# Autodesk Inventor assembly: ASY TKS 3510 Central collector
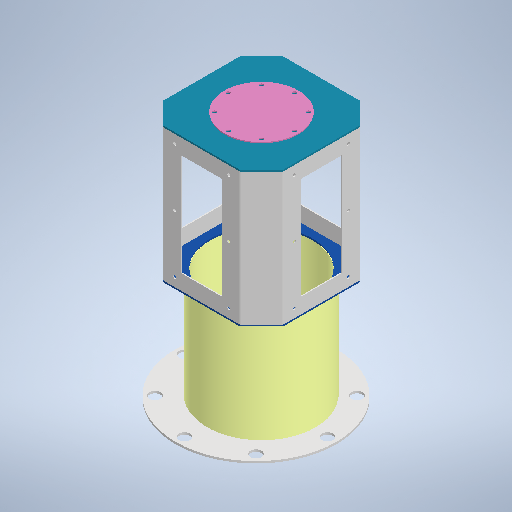
[picture p0: Inventor's stored thumbnail of the model, 512x512]
Saved by Autodesk Inventor 2025 (Build 290162010, 162A)
## iProperties
Created: 2025-07-21
Part Number: ASY TKS 3510 Central collector
Document SubType Name: Assembly
Designer: admin
Author: admin
## Documents named in this file (7)
- C:\Users\pokla\Documents\Inventor\ANP--Antipayuta\FDS 1400\ASY TKS 3510 Central collector.iam
- C:\Users\pokla\Documents\Inventor\ANP--Antipayuta\FDS 1400\ANP 1411 BOTTOM DS main flange.ipt
- C:\Users\pokla\Documents\Inventor\ANP--Antipayuta\FDS 1400\ANP 1452 BOTTOM DS main tube.ipt
- C:\Users\pokla\Documents\Inventor\ANP--Antipayuta\FDS 1400\ANP 1453 BOTTOM DS reduce flange.ipt
- C:\Users\pokla\Documents\Inventor\ANP--Antipayuta\FDS 1400\ANP 1454 BOTTOM DS box wall 1.ipt
- C:\Users\pokla\Documents\Inventor\ANP--Antipayuta\FDS 1400\ANP 1455 BOTTOM DS cup.ipt
- C:\Users\pokla\Documents\Inventor\ANP--Antipayuta\FDS 1400\ANP 1456 BOTTOM DS cup plug.ipt
## Components (7 placed, 6 different names)
1. ANP 1411 BOTTOM DS main flange.ipt:1
2. ANP 1452 BOTTOM DS main tube.ipt:1 — Rigid:6
3. ANP 1453 BOTTOM DS reduce flange.ipt:1 — Rigid:2, Rigid:3, Rigid:6
4. ANP 1454 BOTTOM DS box wall 1.ipt:1 — Rigid:3
5. ANP 1454 BOTTOM DS box wall 1.ipt:2 — Rigid:2, Rigid:5
6. ANP 1455 BOTTOM DS cup.ipt:1 — Rigid:4, Rigid:5
7. ANP 1456 BOTTOM DS cup plug.ipt:1 — Rigid:4
## Relationships (5: WeldJoint 5)
- Rigid:2 [WeldJoint]: ANP 1453 BOTTOM DS reduce flange.ipt:1 ↔ ANP 1454 BOTTOM DS box wall 1.ipt:2
- Rigid:3 [WeldJoint]: ANP 1453 BOTTOM DS reduce flange.ipt:1 ↔ ANP 1454 BOTTOM DS box wall 1.ipt:1
- Rigid:4 [WeldJoint]: ANP 1455 BOTTOM DS cup.ipt:1 ↔ ANP 1456 BOTTOM DS cup plug.ipt:1
- Rigid:5 [WeldJoint]: ANP 1454 BOTTOM DS box wall 1.ipt:2 ↔ ANP 1455 BOTTOM DS cup.ipt:1
- Rigid:6 [WeldJoint]: ANP 1452 BOTTOM DS main tube.ipt:1 ↔ ANP 1453 BOTTOM DS reduce flange.ipt:1
